# Autodesk Inventor assembly: assembly_encoder_coupling
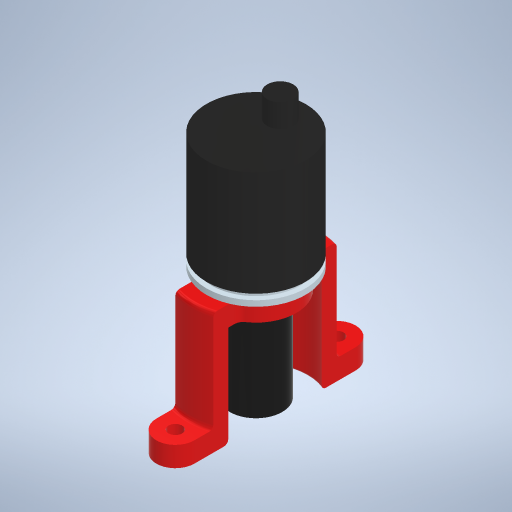
[picture p0: Inventor's stored thumbnail of the model, 512x512]
Saved by Autodesk Inventor 2023 (Build 270158000, 158)
## iProperties
Created: 2023-01-29
Part Number: assembly_encoder_coupling
Document SubType Name: Assembly
Designer: blueh
Author: blueh
## Documents named in this file (4)
- C:\Users\blueh\OneDrive\デスクトップ\2023NHK_RR_1stvid\000_parts_zegi\encoder\assembly_encoder_coupling.iam
- C:\Users\blueh\OneDrive\デスクトップ\2023NHK_RR_1stvid\000_parts_zegi\encoder\Th_3D_hn_1.ipt
- C:\Users\blueh\OneDrive\デスクトップ\2023NHK_RR_1stvid\000_parts_zegi\encoder\encoder v2.ipt
- C:\Users\blueh\OneDrive\デスクトップ\2023NHK_RR_1stvid\000_parts_zegi\encoder\coupling_encoder.ipt
## Components (3 placed, 3 different names)
1. Th_3D_hn_1:1
2. encoder v2:1
3. coupling_encoder:1
## Relationships (2: Insert 2)
- [Insert]: Th_3D_hn_1:1 ↔ encoder v2:1
- [Insert] (-5 mm): encoder v2:1 ↔ coupling_encoder:1
## Named parameters: d570_d504_d485 = 0 mm
